# Autodesk Inventor assembly: 조립품31
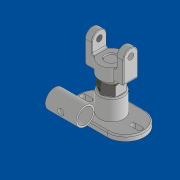
[picture p0: Inventor's stored thumbnail of the model, 180x180]
Saved by Autodesk Inventor 2022 (Build 260153000, 153)
## iProperties
Created: 2022-09-19
Part Number: 조립품31
Document SubType Name: Assembly
Designer: USER
Author: USER
## Documents named in this file (6)
- C:\Users\USER\Desktop\정현서\조립품31.iam
- C:\Users\USER\Desktop\정현서\부품1.ipt
- C:\Users\USER\Desktop\정현서\부품2.ipt
- C:\Users\USER\Desktop\정현서\부품3.ipt
- C:\Users\USER\Desktop\정현서\부품4.ipt
- C:\Users\USER\Documents\Inventor\Content Center Files\R2022\ko-KR\KS B 1012  S1 F\KS B 1012 - M 20(1) F.ipt
## Components (5 placed, 5 different names)
1. 부품1:1 — 삽입:1
2. 부품2:1 — 삽입:3
3. 부품3:1 — 삽입:2, 삽입:3
4. 부품4:1
5. KS B 1012 스타일 1 다듬질 - 미터 M 20:1 — 삽입:1, 삽입:2
## Relationships (3: Insert 3)
- 삽입:1 [Insert]: 부품1:1 ↔ KS B 1012 스타일 1 다듬질 - 미터 M 20:1
- 삽입:2 [Insert]: 부품3:1 ↔ KS B 1012 스타일 1 다듬질 - 미터 M 20:1
- 삽입:3 [Insert]: 부품2:1 ↔ 부품3:1
